# Autodesk Inventor assembly: 1000_Bias_Coil_Spacers_MPSv2_v1
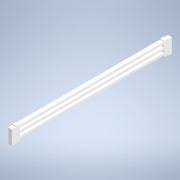
[picture p0: Inventor's stored thumbnail of the model, 180x180]
Saved by Autodesk Inventor 2021 (Build 250183000, 183)
## iProperties
Created: 2020-11-17
Part Number: 1000_Bias_Coil_Spacers_MPSv2_v1
Document SubType Name: Assembly
Designer: Admin
Author: Admin
## Documents named in this file (2)
- C:\Users\Admin\Dropbox (MIT)\MPI Group Folder\MPS\Inventor_Parts\MPSV2\1xxx Assemblies\10xx_Coil_Positioning_Assemblies\1000_Bias_Coil_Spacers_MPSv2_v1.iam
- C:\Users\Admin\Dropbox (MIT)\MPI Group Folder\MPS\Inventor_Parts\MPSV2\4xxx Bias Coil\41xx_Bias_Coils\4100_Bias_Coil_Spacer_MPSv2_v1.ipt
## Components (3 placed, 1 different names)
1. 4100_Bias_Coil_Spacer_MPSv2_v1:1 — Mate:1, Flush:1, Flush:2
2. 4100_Bias_Coil_Spacer_MPSv2_v1:2 — Mate:2, Flush:3, Flush:4
3. 4100_Bias_Coil_Spacer_MPSv2_v1:3 — Mate:1, Flush:1, Flush:2, Mate:2, Flush:3, Flush:4
## Relationships (6: Flush 4, Mate 2)
- Mate:1: 4100_Bias_Coil_Spacer_MPSv2_v1:1 ↔ 4100_Bias_Coil_Spacer_MPSv2_v1:3
- Flush:1: 4100_Bias_Coil_Spacer_MPSv2_v1:1 ↔ 4100_Bias_Coil_Spacer_MPSv2_v1:3
- Flush:2: 4100_Bias_Coil_Spacer_MPSv2_v1:1 ↔ 4100_Bias_Coil_Spacer_MPSv2_v1:3
- Mate:2: 4100_Bias_Coil_Spacer_MPSv2_v1:2 ↔ 4100_Bias_Coil_Spacer_MPSv2_v1:3
- Flush:3: 4100_Bias_Coil_Spacer_MPSv2_v1:2 ↔ 4100_Bias_Coil_Spacer_MPSv2_v1:3
- Flush:4: 4100_Bias_Coil_Spacer_MPSv2_v1:2 ↔ 4100_Bias_Coil_Spacer_MPSv2_v1:3
